# Autodesk Inventor assembly: assembly
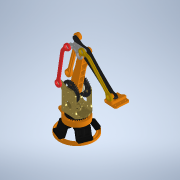
[picture p0: Inventor's stored thumbnail of the model, 180x180]
Saved by Autodesk Inventor 2020 (Build 240168000, 168)
## iProperties
Created: 2016-09-30
Part Number: assembly
Document SubType Name: Assembly
Designer: peter
Mass: 349.077 g
Surface Area: 2089.79 cm^2
Volume: 519.441 cm^3
Density: 0.672024 g/cm^3
Sending System: Autodesk Inventor 2017
Preprocessor: ST-DEVELOPER v16.5
Title: C:\Users\Florin\Desktop\assembly.stp
Author: Florin
## Documents named in this file (20)
- C:\Users\peter\OneDrive\Desktop\RobotArm - 5_3_2024\files\assembly.iam
- C:\Users\peter\OneDrive\Desktop\RobotArm - 5_3_2024\files\base_w_hole.ipt
- C:\Users\peter\OneDrive\Desktop\RobotArm - 5_3_2024\files\lowerShank.ipt
- C:\Users\peter\OneDrive\Desktop\RobotArm - 5_3_2024\files\GearSmall.ipt
- C:\Users\peter\OneDrive\Desktop\RobotArm - 5_3_2024\files\lever.ipt
- C:\Users\peter\OneDrive\Desktop\RobotArm - 5_3_2024\files\GearBig_0.20mmTolerance.ipt
- C:\Users\peter\OneDrive\Desktop\RobotArm - 5_3_2024\files\upperShank.ipt
- C:\Users\peter\OneDrive\Desktop\RobotArm - 5_3_2024\files\pleuel.ipt
- C:\Users\peter\OneDrive\Desktop\RobotArm - 5_3_2024\files\triplate.ipt
- C:\Users\peter\OneDrive\Desktop\RobotArm - 5_3_2024\files\manipulator.ipt
- C:\Users\peter\OneDrive\Desktop\RobotArm - 5_3_2024\files\GearRotate_0.20mmTolerance.ipt
- C:\Users\peter\OneDrive\Desktop\RobotArm - 5_3_2024\files\stepper.ipt
- C:\Users\peter\OneDrive\Desktop\RobotArm - 5_3_2024\files\stepper_short.ipt
- C:\Users\peter\OneDrive\Desktop\RobotArm - 5_3_2024\files\socket.ipt
- C:\Users\peter\OneDrive\Desktop\RobotArm - 5_3_2024\files\leg_30mm.ipt
- C:\Users\peter\OneDrive\Desktop\RobotArm - 5_3_2024\files\stabilizer.ipt
- C:\Users\peter\OneDrive\Desktop\RobotArm - 5_3_2024\files\baseRing.ipt
- C:\Users\peter\OneDrive\Desktop\RobotArm - 5_3_2024\files\pleuel_bend.ipt
- C:\Users\peter\OneDrive\Desktop\RobotArm - 5_3_2024\files\stabilizer_endstop.ipt
- C:\Users\peter\OneDrive\Desktop\RobotArm - 5_3_2024\files\gripperDualclaw.iam
## Components (26 placed, 19 different names)
1. base_w_hole:1 — Mate:20, Mate:21, Mate:22, Mate:23, Mate:24, Mate:25, Mate:31, Mate:32, Mate:39, Mate:40, Mate:55, Mate:59, Mate:60, Mate:61, Mate:62, Mate:63, Mate:68
2. lowerShank:1 — Mate:33, Mate:34, Mate:35, Mate:36, Mate:37, Mate:38, Mate:45, Mate:46, Mate:49, Mate:50
3. GearSmall:1
4. lever:1 — Mate:26, Mate:27, Mate:28, Mate:29, Mate:30, Mate:44, Mate:48
5. GearBig_0.20mmTolerance:1 — Mate:26, Mate:27, Mate:28, Mate:29, Mate:30, Mate:31, Mate:32
6. GearBig_0.20mmTolerance:2 — Mate:33, Mate:34, Mate:35, Mate:36, Mate:37, Mate:38, Mate:39, Mate:40
7. upperShank:1 — Mate:45, Mate:46, Mate:47, Mate:51, Mate:52, Mate:67
8. pleuel:1 — Mate:44, Mate:47, Mate:48, Mate:67
9. triplate:1 — Mate:49, Mate:50, Mate:53, Mate:54, Mate:58, Mate:69
10. manipulator:1 — Mate:51, Mate:52, Mate:57, Mate:66
11. GearRotate_0.20mmTolerance:1 — Mate:18, Mate:19, Mate:20, Mate:21, Mate:22, Mate:23, Mate:24, Mate:25
12. stepper:2
13. stepper:1
14. GearSmall:2
15. stepper_short:3
16. GearSmall:3
17. socket:1 — Mate:10, Mate:11, Mate:12, Mate:13, Mate:14, Mate:15, Mate:16, Mate:18, Mate:19, Mate:64, Mate:65
18. leg_30mm:2 — Mate:7, Mate:8, Mate:9, Mate:10, Mate:11, Mate:65
19. leg_30mm:3 — Mate:1, Mate:2, Mate:3, Mate:12, Mate:13, Mate:64
20. leg_30mm:4 — Mate:4, Mate:5, Mate:6, Mate:14, Mate:15, Mate:16
21. stabilizer:1 — Mate:59, Mate:60, Mate:61, Mate:62, Mate:63
22. baseRing:1 — Mate:1, Mate:2, Mate:3, Mate:4, Mate:5, Mate:6, Mate:7, Mate:8, Mate:9
23. pleuel_bend:1 — Mate:53, Mate:57, Mate:58, Mate:66
24. pleuel_bend:2 — Mate:54, Mate:55, Mate:68, Mate:69
25. stabilizer_endstop:1
26. gripperDualclaw:1 [sub-assembly]
## Relationships (64: Mate 64)
- Mate:1: leg_30mm:3 ↔ baseRing:1
- Mate:2: leg_30mm:3 ↔ baseRing:1
- Mate:3: leg_30mm:3 ↔ baseRing:1
- Mate:4: leg_30mm:4 ↔ baseRing:1
- Mate:5: leg_30mm:4 ↔ baseRing:1
- Mate:6: leg_30mm:4 ↔ baseRing:1
- Mate:7: leg_30mm:2 ↔ baseRing:1
- Mate:8: leg_30mm:2 ↔ baseRing:1
- Mate:9: leg_30mm:2 ↔ baseRing:1
- Mate:10: socket:1 ↔ leg_30mm:2
- Mate:11: socket:1 ↔ leg_30mm:2
- Mate:12: socket:1 ↔ leg_30mm:3
- Mate:13: socket:1 ↔ leg_30mm:3
- Mate:14: socket:1 ↔ leg_30mm:4
- Mate:15: socket:1 ↔ leg_30mm:4
- Mate:16: socket:1 ↔ leg_30mm:4
- Mate:18: GearRotate_0.20mmTolerance:1 ↔ socket:1
- Mate:19: GearRotate_0.20mmTolerance:1 ↔ socket:1
- Mate:20: base_w_hole:1 ↔ GearRotate_0.20mmTolerance:1
- Mate:21: base_w_hole:1 ↔ GearRotate_0.20mmTolerance:1
- Mate:22: base_w_hole:1 ↔ GearRotate_0.20mmTolerance:1
- Mate:23: base_w_hole:1 ↔ GearRotate_0.20mmTolerance:1
- Mate:24: base_w_hole:1 ↔ GearRotate_0.20mmTolerance:1
- Mate:25: base_w_hole:1 ↔ GearRotate_0.20mmTolerance:1
- Mate:26: lever:1 ↔ GearBig_0.20mmTolerance:1
- Mate:27: lever:1 ↔ GearBig_0.20mmTolerance:1
- Mate:28: lever:1 ↔ GearBig_0.20mmTolerance:1
- Mate:29: lever:1 ↔ GearBig_0.20mmTolerance:1
- Mate:30: lever:1 ↔ GearBig_0.20mmTolerance:1
- Mate:31: base_w_hole:1 ↔ GearBig_0.20mmTolerance:1
- Mate:32: base_w_hole:1 ↔ GearBig_0.20mmTolerance:1
- Mate:33: lowerShank:1 ↔ GearBig_0.20mmTolerance:2
- Mate:34: lowerShank:1 ↔ GearBig_0.20mmTolerance:2
- Mate:35: lowerShank:1 ↔ GearBig_0.20mmTolerance:2
- Mate:36: lowerShank:1 ↔ GearBig_0.20mmTolerance:2
- Mate:37: lowerShank:1 ↔ GearBig_0.20mmTolerance:2
- Mate:38: lowerShank:1 ↔ GearBig_0.20mmTolerance:2
- Mate:39: base_w_hole:1 ↔ GearBig_0.20mmTolerance:2
- Mate:40: base_w_hole:1 ↔ GearBig_0.20mmTolerance:2
- Mate:44: lever:1 ↔ pleuel:1
- Mate:45: lowerShank:1 ↔ upperShank:1
- Mate:46: lowerShank:1 ↔ upperShank:1
- Mate:47: upperShank:1 ↔ pleuel:1
- Mate:48: lever:1 ↔ pleuel:1
- Mate:49: lowerShank:1 ↔ triplate:1
- Mate:50: lowerShank:1 ↔ triplate:1
- Mate:51: upperShank:1 ↔ manipulator:1
- Mate:52: upperShank:1 ↔ manipulator:1
- Mate:53: triplate:1 ↔ pleuel_bend:1
- Mate:54: triplate:1 ↔ pleuel_bend:2
- Mate:55: base_w_hole:1 ↔ pleuel_bend:2
- Mate:57: manipulator:1 ↔ pleuel_bend:1
- Mate:58: triplate:1 ↔ pleuel_bend:1
- Mate:59: base_w_hole:1 ↔ stabilizer:1
- Mate:60: base_w_hole:1 ↔ stabilizer:1
- Mate:61: base_w_hole:1 ↔ stabilizer:1
- Mate:62: base_w_hole:1 ↔ stabilizer:1
- Mate:63: base_w_hole:1 ↔ stabilizer:1
- Mate:64: socket:1 ↔ leg_30mm:3
- Mate:65: socket:1 ↔ leg_30mm:2
- Mate:66: manipulator:1 ↔ pleuel_bend:1
- Mate:67: upperShank:1 ↔ pleuel:1
- Mate:68: base_w_hole:1 ↔ pleuel_bend:2
- Mate:69: triplate:1 ↔ pleuel_bend:2
